# Autodesk Inventor assembly: roller assembly
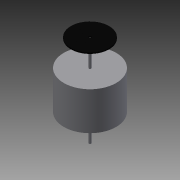
[picture p0: Inventor's stored thumbnail of the model, 180x180]
Saved by Autodesk Inventor 2015 (Build 190159000, 159)
## iProperties
Created: 2014-11-08
Part Number: roller assembly
Document SubType Name: Assembly
Designer: jesse
Author: jesse
## Documents named in this file (4)
- C:\Users\jesse\Desktop\robot\arm\roller assembly.iam
- C:\Users\jesse\Desktop\robot\arm\foam gripper2.ipt
- C:\Users\jesse\Desktop\robot\arm\roller.ipt
- C:\Users\jesse\Desktop\robot\arm\rotating rod.ipt
## Components (3 placed, 3 different names)
1. foam gripper2:1 — Mate:2, Mate:3
2. roller:1 — Mate:2
3. rotating rod:1 — Mate:3
## Relationships (2: Mate 2)
- Mate:2: foam gripper2:1 ↔ roller:1
- Mate:3: foam gripper2:1 ↔ rotating rod:1
